# Autodesk Inventor assembly: Lath
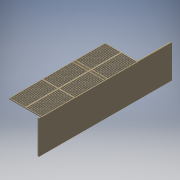
[picture p0: Inventor's stored thumbnail of the model, 180x180]
Saved by Autodesk Inventor 2018 (Build 220112000, 112)
## iProperties
Created: 2019-05-10
Part Number: Lath
Document SubType Name: Assembly
Designer: 10043883
Author: 10043883
## Documents named in this file (5)
- C:\Users\10043883\Documents\GitHub\IED-files\Lath.iam
- C:\Users\10043883\Documents\GitHub\IED-files\Lathhouse\Lathhouse wall.ipt
- C:\Users\10043883\Documents\GitHub\IED-files\Foor.ipt
- C:\Users\10043883\Documents\GitHub\IED-files\Foor_MIR.ipt
- C:\Users\10043883\Documents\GitHub\IED-files\Lathhouse\Lathhouse wall_MIR.ipt
## Components (8 placed, 4 different names)
1. Foor:1 — Mate:1
2. Lathhouse wall:1 — Mate:1, Mate:2, Mate:5, Mate:6
3. Lathhouse wall:2 — Mate:2
4. Foor_MIR:1 — Mate:3
5. Lathhouse wall_MIR:1 — Mate:3, Mate:4
6. Lathhouse wall_MIR:2 — Mate:4
7. Lathhouse wall:3 — Mate:5
8. Lathhouse wall:4 — Mate:6
## Relationships (6: Mate 6)
- Mate:1: Foor:1 ↔ Lathhouse wall:1
- Mate:2: Lathhouse wall:1 ↔ Lathhouse wall:2
- Mate:3: Foor_MIR:1 ↔ Lathhouse wall_MIR:1
- Mate:4: Lathhouse wall_MIR:1 ↔ Lathhouse wall_MIR:2
- Mate:5: Lathhouse wall:1 ↔ Lathhouse wall:3
- Mate:6: Lathhouse wall:1 ↔ Lathhouse wall:4
